# Autodesk Inventor assembly: V6Intake
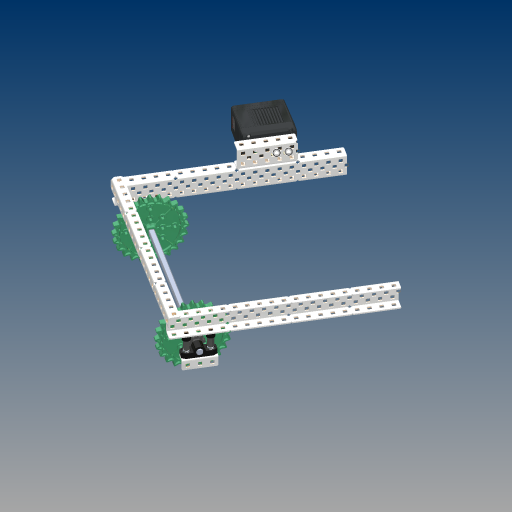
[picture p0: Inventor's stored thumbnail of the model, 512x512]
Saved by Autodesk Inventor 2023 (Build 270158000, 158)
## iProperties
Created: 2024-03-10
Part Number: V6Intake
Document SubType Name: Assembly
Designer: eddie
Author: eddie
## Documents named in this file (19)
- C:\Users\eddie\Documents\81208X-Over-Under-CAD\V6\V6Intake.iam
- C:\Users\eddie\Documents\81208X-Over-Under-CAD\VEX-CAD-Inventor-1.4.0\Structure\C Channel\Aluminum 1x2x1\Alu C 1x2x1x19.ipt
- C:\Users\eddie\Documents\81208X-Over-Under-CAD\VEX-CAD-Inventor-1.4.0\Structure\Angle\Aluminum\1x1\Alu Angle 1x1x20.ipt
- C:\Users\eddie\Documents\81208X-Over-Under-CAD\VEX-CAD-Inventor-1.4.0\Structure\Angle\Aluminum\1x1\Alu Angle 1x1x3.ipt
- C:\Users\eddie\Documents\81208X-Over-Under-CAD\VEX-CAD-Inventor-1.4.0\Motion\Spacers\Spacer Nylon .375 OD\NSpacer .375 OD x .250.ipt
- C:\Users\eddie\Documents\81208X-Over-Under-CAD\VEX-CAD-Inventor-1.4.0\Motion\Spacers\Spacer Nylon .375 OD.ipt
- C:\Users\eddie\Documents\81208X-Over-Under-CAD\VEX-CAD-Inventor-1.4.0\Structure\Standoff\Standoff .50.ipt
- C:\Users\eddie\Documents\81208X-Over-Under-CAD\VEX-CAD-Inventor-1.4.0\Structure\Standoff.ipt
- C:\Users\eddie\Documents\81208X-Over-Under-CAD\VEX-CAD-Inventor-1.4.0\Motion\Shaft HS\HS Pillow Bearing Block.ipt
- C:\Users\eddie\Documents\81208X-Over-Under-CAD\VEX-CAD-Inventor-1.4.0\Structure\Hardware\Nut Nylock.ipt
- C:\Users\eddie\Documents\81208X-Over-Under-CAD\VEX-CAD-Inventor-1.4.0\Motion\Shaft HS\Shaft HS\Shaft HS 10.0 in.ipt
- C:\Users\eddie\Documents\81208X-Over-Under-CAD\VEX-CAD-Inventor-1.4.0\Motion\Shaft HS\Shaft HS.ipt
- C:\Users\eddie\Documents\81208X-Over-Under-CAD\VEX-CAD-Inventor-1.4.0\Motion\Sprockets\6P Sprocket\6P 8T Sprocket, Square.iam
- C:\Users\eddie\Documents\81208X-Over-Under-CAD\VEX-CAD-Inventor-1.4.0\Motion\Sprockets\6P Sprocket.iam
- C:\Users\eddie\Documents\81208X-Over-Under-CAD\VEX-CAD-Inventor-1.4.0\Motion\Sprockets\9P Sprocket\9P 24T Sprocket, Square.iam
- C:\Users\eddie\Documents\81208X-Over-Under-CAD\VEX-CAD-Inventor-1.4.0\Motion\Sprockets\9P Sprocket.iam
- C:\Users\eddie\Documents\81208X-Over-Under-CAD\VEX-CAD-Inventor-1.4.0\Structure\C Channel\Aluminum 1x2x1\Alu C 1x2x1x5.ipt
- C:\Users\eddie\Documents\81208X-Over-Under-CAD\VEX-CAD-Inventor-1.4.0\Electronics\V5 Motor.ipt
- C:\Users\eddie\Documents\81208X-Over-Under-CAD\VEX-CAD-Inventor-1.4.0\Structure\Plate\Aluminum\Alu Plate 1x20.ipt
## Components (27 placed, 13 different names)
1. Alu C 1x2x1x19:1 — Insert:2, Insert:5, Insert:6, Insert:31, Insert:32, Insert:35
2. Alu C 1x2x1x19:2 — Insert:1, Insert:3, Insert:4, Insert:34
3. Alu Angle 1x1x20:1 — Insert:1, Insert:2
4. Alu Angle 1x1x3:1 — Insert:17, Insert:18
5. Alu Angle 1x1x3:2 — Insert:23, Insert:24
6. NSpacer .375 OD x .250:1 — Insert:3, Insert:8
7. NSpacer .375 OD x .250:2 — Insert:4, Insert:7
8. NSpacer .375 OD x .250:3 — Insert:5, Insert:9
9. NSpacer .375 OD x .250:4 — Insert:6, Insert:10
10. Standoff .50:1 — Insert:8, Insert:16
11. Standoff .50:2 — Insert:7, Insert:15
12. Standoff .50:3 — Insert:9, Insert:19
13. Standoff .50:4 — Insert:10, Insert:21
14. HS Pillow Bearing Block:1 — Insert:11, Insert:12, Insert:17, Insert:18, Insert:25
15. HS Pillow Bearing Block:2 — Insert:13, Insert:14, Insert:23, Insert:24
16. Nut Nylock:1 — Insert:12, Insert:16
17. Nut Nylock:2 — Insert:11, Insert:15
18. Nut Nylock:3 — Insert:14, Insert:19
19. Nut Nylock:4 — Insert:13, Insert:21
20. Shaft HS 10.0 in:1 — Insert:25, Insert:27, Insert:28
21. 6P 8T Sprocket, Square:2 [sub-assembly] — Insert:27, Insert:30
22. 6P 8T Sprocket, Square:3 [sub-assembly] — Insert:28, Insert:29
23. 9P 24T Sprocket, Square:1 [sub-assembly] — Insert:29
24. 9P 24T Sprocket, Square:2 [sub-assembly] — Insert:30
25. Alu C 1x2x1x5:1 — Insert:31, Insert:32, Insert:33
26. V5 Motor:2 — Insert:33
27. Alu Plate 1x20:1 — Insert:34, Insert:35
## Relationships (32: Insert 32)
- Insert:1: Alu C 1x2x1x19:2 ↔ Alu Angle 1x1x20:1
- Insert:2: Alu C 1x2x1x19:1 ↔ Alu Angle 1x1x20:1
- Insert:3: Alu C 1x2x1x19:2 ↔ NSpacer .375 OD x .250:1
- Insert:4: Alu C 1x2x1x19:2 ↔ NSpacer .375 OD x .250:2
- Insert:5: Alu C 1x2x1x19:1 ↔ NSpacer .375 OD x .250:3
- Insert:6: Alu C 1x2x1x19:1 ↔ NSpacer .375 OD x .250:4
- Insert:7: NSpacer .375 OD x .250:2 ↔ Standoff .50:2
- Insert:8: NSpacer .375 OD x .250:1 ↔ Standoff .50:1
- Insert:9: NSpacer .375 OD x .250:3 ↔ Standoff .50:3
- Insert:10: NSpacer .375 OD x .250:4 ↔ Standoff .50:4
- Insert:11: HS Pillow Bearing Block:1 ↔ Nut Nylock:2
- Insert:12: HS Pillow Bearing Block:1 ↔ Nut Nylock:1
- Insert:13: HS Pillow Bearing Block:2 ↔ Nut Nylock:4
- Insert:14: HS Pillow Bearing Block:2 ↔ Nut Nylock:3
- Insert:15: Standoff .50:2 ↔ Nut Nylock:2
- Insert:16: Standoff .50:1 ↔ Nut Nylock:1
- Insert:17: Alu Angle 1x1x3:1 ↔ HS Pillow Bearing Block:1
- Insert:18: Alu Angle 1x1x3:1 ↔ HS Pillow Bearing Block:1
- Insert:19: Standoff .50:3 ↔ Nut Nylock:3
- Insert:21: Standoff .50:4 ↔ Nut Nylock:4
- Insert:23: Alu Angle 1x1x3:2 ↔ HS Pillow Bearing Block:2
- Insert:24: Alu Angle 1x1x3:2 ↔ HS Pillow Bearing Block:2
- Insert:25: HS Pillow Bearing Block:1 ↔ Shaft HS 10.0 in:1
- Insert:27: Shaft HS 10.0 in:1 ↔ 6P 8T Sprocket, Square:2
- Insert:28: Shaft HS 10.0 in:1 ↔ 6P 8T Sprocket, Square:3
- Insert:29: 6P 8T Sprocket, Square:3 ↔ 9P 24T Sprocket, Square:1
- Insert:30: 6P 8T Sprocket, Square:2 ↔ 9P 24T Sprocket, Square:2
- Insert:31: Alu C 1x2x1x19:1 ↔ Alu C 1x2x1x5:1
- Insert:32: Alu C 1x2x1x19:1 ↔ Alu C 1x2x1x5:1
- Insert:33: Alu C 1x2x1x5:1 ↔ V5 Motor:2
- Insert:34: Alu C 1x2x1x19:2 ↔ Alu Plate 1x20:1
- Insert:35: Alu C 1x2x1x19:1 ↔ Alu Plate 1x20:1
